# Autodesk Inventor assembly: Baugruppe1
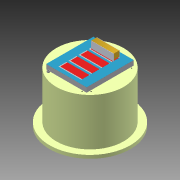
[picture p0: Inventor's stored thumbnail of the model, 180x180]
Saved by Autodesk Inventor 2013 (Build 170138000, 138)
## iProperties
Created: 2014-01-06
Part Number: Baugruppe1
Document SubType Name: Assembly
Designer: Frank Meier
Author: Frank Meier
## Documents named in this file (4)
- C:\Users\Frank Meier\Documents\Inventor\Delvotec-Saugplatte\Baugruppe1.iam
- C:\Users\Frank Meier\Documents\Inventor\Delvotec-Saugplatte\Chuck4modules.iam
- C:\Users\Frank Meier\Documents\Inventor\Delvotec-Saugplatte\SuctionblockDelcotec.iam
- C:\Users\Frank Meier\Documents\Inventor\Delvotec-Saugplatte\HDI-Niederdrücker.iam
## Components (3 placed, 3 different names)
1. Chuck4modules:1 [sub-assembly] — Passend:1, Tangential:1, Tangential:2, Tangential:3, Passend:2, Fluchtend:1, Fluchtend:2
2. SuctionblockDelcotec:1 [sub-assembly] — Passend:1, Tangential:1, Tangential:2, Tangential:3
3. HDI-Niederdrücker:1 [sub-assembly] — Passend:2, Fluchtend:1, Fluchtend:2
## Relationships (7: Tangent 3, Mate 2, Flush 2)
- Passend:1 [Mate]: Chuck4modules:1 ↔ SuctionblockDelcotec:1
- Tangential:1: Chuck4modules:1 ↔ SuctionblockDelcotec:1
- Tangential:2: Chuck4modules:1 ↔ SuctionblockDelcotec:1
- Tangential:3: Chuck4modules:1 ↔ SuctionblockDelcotec:1
- Passend:2 [Mate]: Chuck4modules:1 ↔ HDI-Niederdrücker:1
- Fluchtend:1 [Flush] (1.78 mm): Chuck4modules:1 ↔ HDI-Niederdrücker:1
- Fluchtend:2 [Flush] (-1.415 mm): Chuck4modules:1 ↔ HDI-Niederdrücker:1
